# Autodesk Inventor assembly: structure
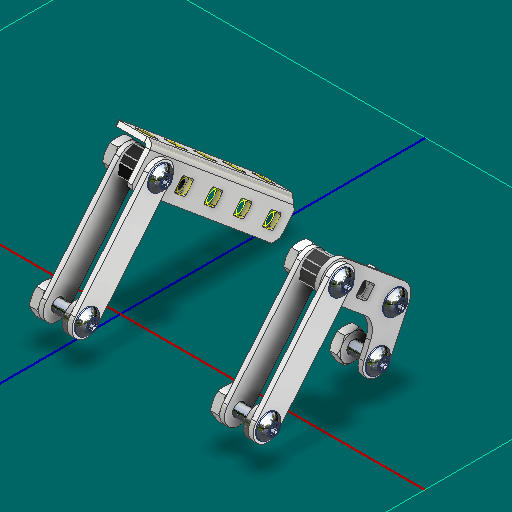
[picture p0: Inventor's stored thumbnail of the model, 512x512]
Saved by Autodesk Inventor 2025 (Build 290162000, 162)
## iProperties
Created: 2024-08-16
Part Number: structure
Document SubType Name: Assembly
Designer: averey
Author: averey
## Documents named in this file (14)
- C:\Users\avere\vex_robotics_high_stakes\hardware\cad\ATLAS\chassis\drive_pod\gearbox\structure.iam
- C:\Users\avere\vex_robotics_high_stakes\hardware\cad\VEX-CAD-Inventor\Structure\Angle\Aluminum 1x1\Alu Angle 1x1x5.ipt
- C:\Users\avere\vex_robotics_high_stakes\hardware\cad\ATLAS\chassis\drive_pod\gearbox\custom_parts\straight_gusset.ipt
- C:\Users\avere\vex_robotics_high_stakes\hardware\cad\custom_parts\modified_parts\Bearing Flat Low Profile 2-Hole.ipt
- C:\Users\avere\vex_robotics_high_stakes\hardware\cad\VEX-CAD-Inventor\Motion\Shaft LS\Bearing Flat Low Profile.ipt
- C:\Users\avere\vex_robotics_high_stakes\hardware\cad\VEX-CAD-Inventor\Structure\Hardware\Screw Steel - Star\SScrew Star Smooth .625.ipt
- C:\Users\avere\vex_robotics_high_stakes\hardware\cad\VEX-CAD-Inventor\Structure\Hardware\Screw Steel - Star.ipt
- C:\Users\avere\vex_robotics_high_stakes\hardware\cad\VEX-CAD-Inventor\Structure\Hardware\Nut Nylon\Nut Nylon - White.ipt
- C:\Users\avere\vex_robotics_high_stakes\hardware\cad\VEX-CAD-Inventor\Structure\Hardware\Nut Nylon.ipt
- C:\Users\avere\vex_robotics_high_stakes\hardware\cad\VEX-CAD-Inventor\Motion\Spacers\Washer Steel\SWasher .375 OD x .062500.ipt
- C:\Users\avere\vex_robotics_high_stakes\hardware\cad\VEX-CAD-Inventor\Motion\Spacers\Washer Steel.ipt
- C:\Users\avere\vex_robotics_high_stakes\hardware\cad\VEX-CAD-Inventor\Structure\Hardware\Screw Shoulder Robosource\SScrew Shoulder Smooth .500 x .04.ipt
- C:\Users\avere\vex_robotics_high_stakes\hardware\cad\VEX-CAD-Inventor\Structure\Hardware\Screw Shoulder Robosource.ipt
- C:\Users\avere\vex_robotics_high_stakes\hardware\cad\ATLAS\chassis\drive_pod\gearbox\custom_parts\bent_gusset_improved.ipt
## Components (22 placed, 9 different names)
1. Alu Angle 1x1x5:1 — Insert:1, Insert:2, Mate:3, Mate:11
2. straight_gusset:1 — Insert:1, Mate:1, Mate:2, Insert:3, Mate:8, Insert:6, Insert:7, Insert:19
3. straight_gusset:2 — Mate:1, Mate:2, Mate:4, Insert:10, Insert:11
4. Bearing Flat Low Profile 2-Hole:1 — Insert:2, Mate:3, Mate:4
5. straight_gusset:3 — Mate:7, Insert:8, Insert:9, Insert:18, Insert:20, Angle:1
6. straight_gusset:4 — Insert:3, Mate:7, Mate:8, Insert:12, Insert:13
7. Bearing Flat Low Profile:1 — Insert:16, Insert:17, Mate:9, Mate:10, Mate:11
8. SScrew Star Smooth .625:1 — Insert:7
9. SScrew Star Smooth .625:2 — Insert:6
10. SScrew Star Smooth .625:3 — Insert:8
11. SScrew Star Smooth .625:4 — Insert:9, Mate:9
12. Nut Nylon - White:1 — Insert:11
13. Nut Nylon - White:2 — Insert:10
14. Nut Nylon - White:3 — Insert:13
15. Nut Nylon - White:4 — Insert:12
16. SWasher .375 OD x .062500:1 — Insert:18
17. SWasher .375 OD x .062500:2 — Insert:19
18. SScrew Shoulder Smooth .500 x .04:1 — Insert:16, Insert:21
19. Nut Nylon - White:5 — Insert:17
20. SScrew Shoulder Smooth .500 x .04:2 — Insert:22
21. Nut Nylon - White:6 — Insert:23
22. bent_gusset_improved:1 — Insert:20, Mate:10, Insert:21, Insert:22, Insert:23, Angle:1
## Relationships (31: Insert 19, Mate 11, Angle 1)
- Insert:1: Alu Angle 1x1x5:1 ↔ straight_gusset:1
- Mate:1: straight_gusset:1 ↔ straight_gusset:2
- Mate:2: straight_gusset:1 ↔ straight_gusset:2
- Insert:2: Alu Angle 1x1x5:1 ↔ Bearing Flat Low Profile 2-Hole:1
- Mate:3: Alu Angle 1x1x5:1 ↔ Bearing Flat Low Profile 2-Hole:1
- Mate:4: straight_gusset:2 ↔ Bearing Flat Low Profile 2-Hole:1
- [Mate]: straight_gusset:3 ↔ straight_gusset:4
- [Mate]: straight_gusset:3 ↔ straight_gusset:4
- Insert:3 (49.2125 mm): straight_gusset:1 ↔ straight_gusset:4
- Mate:7 (7.9375 mm): straight_gusset:3 ↔ straight_gusset:4
- Mate:8: straight_gusset:1 ↔ straight_gusset:4
- Insert:6: straight_gusset:1 ↔ SScrew Star Smooth .625:2
- Insert:7: straight_gusset:1 ↔ SScrew Star Smooth .625:1
- Insert:8: straight_gusset:3 ↔ SScrew Star Smooth .625:3
- Insert:9: straight_gusset:3 ↔ SScrew Star Smooth .625:4
- Insert:10: straight_gusset:2 ↔ Nut Nylon - White:2
- Insert:11: straight_gusset:2 ↔ Nut Nylon - White:1
- Insert:12: straight_gusset:4 ↔ Nut Nylon - White:4
- Insert:13: straight_gusset:4 ↔ Nut Nylon - White:3
- Insert:16 (1.5875 mm): Bearing Flat Low Profile:1 ↔ SScrew Shoulder Smooth .500 x .04:1
- Insert:17 (1.27 mm): Bearing Flat Low Profile:1 ↔ Nut Nylon - White:5
- Insert:18: straight_gusset:3 ↔ SWasher .375 OD x .062500:1
- Insert:19: straight_gusset:1 ↔ SWasher .375 OD x .062500:2
- Insert:20: straight_gusset:3 ↔ bent_gusset_improved:1
- Mate:9: Bearing Flat Low Profile:1 ↔ SScrew Star Smooth .625:4
- Mate:10: Bearing Flat Low Profile:1 ↔ bent_gusset_improved:1
- Insert:21: SScrew Shoulder Smooth .500 x .04:1 ↔ bent_gusset_improved:1
- Insert:22: SScrew Shoulder Smooth .500 x .04:2 ↔ bent_gusset_improved:1
- Mate:11: Alu Angle 1x1x5:1 ↔ Bearing Flat Low Profile:1
- Insert:23 (6.35 mm): Nut Nylon - White:6 ↔ bent_gusset_improved:1
- Angle:1 (-90.0274 deg): straight_gusset:3 ↔ bent_gusset_improved:1
## Named parameters: d15_d3 = 0 mm, d16_d4 = 0 mm
